# Autodesk Inventor assembly: OUTK_000_Assembly
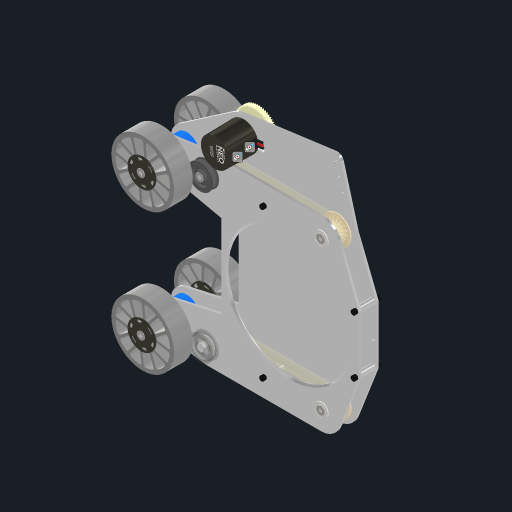
[picture p0: Inventor's stored thumbnail of the model, 512x512]
Saved by Autodesk Inventor 2024.2 (Build 282272000, 272)
## iProperties
Created: 2024-11-24
Part Number: OUTK_000_Assembly
Document SubType Name: Assembly
Designer: Bryan
Mass: 9682.5 g
Surface Area: 20203.5 cm^2
Volume: 5331.75 cm^3
Author: Bryan
## Documents named in this file (25)
- C:\Users\bobsb\OneDrive\Documents\GitHub\1622-2024-Casino-Clash-CAD-A-Thon\Outtake\OUTK_000_Assembly.iam
- C:\Users\bobsb\OneDrive\Documents\GitHub\1622-2024-Casino-Clash-CAD-A-Thon\Outtake\OUTK_002_ShotPlateNoReceptacle.ipt
- C:\Users\bobsb\OneDrive\Documents\GitHub\1622-2024-Casino-Clash-CAD-A-Thon\Outtake\OUTK_002_ShotPlateReceptacle.ipt
- C:\Users\bobsb\OneDrive\Documents\GitHub\1622-2024-Casino-Clash-CAD-A-Thon\COTS Library\Motion\Bearings\COTS_WCP-0783_1.125ODHexBearing.ipt
- C:\Users\bobsb\OneDrive\Documents\GitHub\1622-2024-Casino-Clash-CAD-A-Thon\COTS Library\Motion\Wheels\Compliant Wheels\5in compliant wheels\COTS_5 Straight Flex Wheel (.ipt
- C:\Users\bobsb\OneDrive\Documents\GitHub\1622-2024-Casino-Clash-CAD-A-Thon\COTS Library\Adapters\COTS_1_2” Hex Bore Aluminum VersaHub (217-2592)(1).ipt
- C:\Users\bobsb\OneDrive\Documents\GitHub\1622-2024-Casino-Clash-CAD-A-Thon\COTS Library\Motion\Wheels\Compliant Wheels\2in compliant wheels\0.500in hex bore\COTS_am-3462_2indiameter_0.500inhexbore_durometer50A_CompliantWheel.ipt
- C:\Users\bobsb\OneDrive\Documents\GitHub\1622-2024-Casino-Clash-CAD-A-Thon\Outtake\OUTK_010_Grippy.ipt
- C:\Users\bobsb\OneDrive\Documents\GitHub\1622-2024-Casino-Clash-CAD-A-Thon\Outtake\OUTK_011_Tubing.ipt
- C:\Users\bobsb\OneDrive\Documents\GitHub\1622-2024-Casino-Clash-CAD-A-Thon\COTS Library\Fasteners\Bolts\Set Screws\10-32\COTS_91375A446_Alloy Steel Cup-Point Set Screw.ipt
- C:\Users\bobsb\OneDrive\Documents\GitHub\1622-2024-Casino-Clash-CAD-A-Thon\COTS Library\Motion\Pulleys\HTD5M\10mm Wide\COTS_30T_WCP-0565.ipt
- C:\Users\bobsb\OneDrive\Documents\GitHub\1622-2024-Casino-Clash-CAD-A-Thon\COTS Library\Motors\COTS_REV-21-1650-V1.1_Neo1.1.ipt
- C:\Users\bobsb\OneDrive\Documents\GitHub\1622-2024-Casino-Clash-CAD-A-Thon\COTS Library\Fasteners\Bolts\Button-Head\10-32\COTS_91255A265_Button Head Hex Drive Screw.ipt
- C:\Users\bobsb\OneDrive\Documents\GitHub\1622-2024-Casino-Clash-CAD-A-Thon\COTS Library\Adapters\COTS_REV-21-1879_8mmKeyTo0.5Hex.ipt
- C:\Users\bobsb\OneDrive\Documents\GitHub\1622-2024-Casino-Clash-CAD-A-Thon\COTS Library\Motion\Pulleys\HTD5M\10mm Wide\COTS_24T_WCP-0564.ipt
- C:\Users\bobsb\OneDrive\Documents\GitHub\1622-2024-Casino-Clash-CAD-A-Thon\COTS Library\Motion\Gears\20DP gears\Aluminum\0.5in hex\COTS_60T_WCP-0720(1).ipt
- C:\Users\bobsb\OneDrive\Documents\GitHub\1622-2024-Casino-Clash-CAD-A-Thon\Outtake\OUTK_012_Spacer1.ipt
- C:\Users\bobsb\OneDrive\Documents\GitHub\1622-2024-Casino-Clash-CAD-A-Thon\Outtake\OUTK_013_Standoff1.ipt
- C:\Users\bobsb\OneDrive\Documents\GitHub\1622-2024-Casino-Clash-CAD-A-Thon\COTS Library\Fasteners\Bolts\Socket-Head\0.25-20\COTS_91251A537_Black-Oxide Alloy Steel Socket Head Screw_.25-20_.5in.ipt
- C:\Users\bobsb\OneDrive\Documents\GitHub\1622-2024-Casino-Clash-CAD-A-Thon\Outtake\OUTK_014_Shaft1.ipt
- C:\Users\bobsb\OneDrive\Documents\GitHub\1622-2024-Casino-Clash-CAD-A-Thon\Outtake\OUTK_015_Shaft2.ipt
- C:\Users\bobsb\OneDrive\Documents\GitHub\1622-2024-Casino-Clash-CAD-A-Thon\Outtake\OUTK_016_Shaft3.ipt
- C:\Users\bobsb\OneDrive\Documents\GitHub\1622-2024-Casino-Clash-CAD-A-Thon\Outtake\OUTK_016_Shaft4.ipt
- C:\Users\bobsb\OneDrive\Documents\GitHub\1622-2024-Casino-Clash-CAD-A-Thon\Outtake\OUTK_018_Spacer2.ipt
- C:\Users\bobsb\OneDrive\Documents\GitHub\1622-2024-Casino-Clash-CAD-A-Thon\COTS Library\Fasteners\Washers\COTS_90107A029_316 Stainless Steel Washer.ipt
## Components (131 placed, 24 different names)
1. OUTK_002_ShotPlateReceptacle:1 — Mate:141, Mate:179, Mate:183, Mate:185, Mate:190, Mate:205, Mate:207, Mate:208, Mate:210, Mate:211, Mate:212, Mate:213, Mate:225, Mate:228, Mate:229, Mate:232, Mate:244, Mate:245, Mate:246, Mate:247, Mate:249, Mate:251, Mate:252, Mate:253, Mate:254, Mate:255, Mate:262, Mate:267
2. COTS_WCP-0783_1.125ODHexBearing:1 — Mate:72, Mate:107, Mate:166, Mate:168, Mate:204
3. COTS_WCP-0783_1.125ODHexBearing:2 — Mate:74, Mate:106, Mate:108, Mate:145, Mate:205, Mate:208, Mate:235
4. COTS_WCP-0783_1.125ODHexBearing:3 — Mate:120, Mate:143, Mate:146, Mate:229, Mate:232
5. COTS_WCP-0783_1.125ODHexBearing:4 — Mate:124, Mate:230, Mate:231, Mate:269, Flush:24
6. COTS_WCP-0783_1.125ODHexBearing:5 — Mate:117, Mate:225, Mate:228, Flush:21
7. COTS_WCP-0783_1.125ODHexBearing:6 — Mate:123, Mate:226, Mate:227, Mate:258
8. COTS_WCP-0783_1.125ODHexBearing:7 — Mate:122, Mate:160, Mate:200, Mate:222
9. COTS_WCP-0783_1.125ODHexBearing:8 — Mate:71, Mate:110, Mate:111, Mate:163, Mate:165, Mate:215
10. COTS_WCP-0783_1.125ODHexBearing:9 — Mate:119, Mate:142, Mate:144, Mate:267
11. COTS_WCP-0783_1.125ODHexBearing:10 — Mate:73, Mate:112, Mate:139, Mate:140, Mate:207, Mate:213, Mate:214
12. COTS_WCP-0783_1.125ODHexBearing:11 — Mate:121, Mate:223, Mate:224
13. COTS_WCP-0783_1.125ODHexBearing:12 — Mate:118, Mate:197, Flush:18, Mate:262
14. COTS_5 Straight Flex Wheel (:1 — Mate:71, Mate:75, Mate:80, Mate:85, Mate:88, Mate:89, Mate:90
15. COTS_5 Straight Flex Wheel (:2 — Mate:72, Mate:76, Mate:81, Mate:86, Mate:87, Mate:94, Mate:95, Mate:96
16. COTS_5 Straight Flex Wheel (:3 — Mate:73, Mate:78, Mate:79, Mate:84, Mate:91, Mate:92, Mate:93
17. COTS_5 Straight Flex Wheel (:4 — Mate:74, Mate:77, Mate:82, Mate:83, Mate:97, Mate:98, Mate:99
18. COTS_1_2” Hex Bore Aluminum VersaHub (217-2592)(1):1 — Mate:77, Mate:82, Mate:83, Mate:135, Flush:8, Mate:194, Flush:14
19. COTS_1_2” Hex Bore Aluminum VersaHub (217-2592)(1):2 — Mate:76, Mate:81, Mate:86, Mate:87, Mate:130, Flush:3
20. COTS_1_2” Hex Bore Aluminum VersaHub (217-2592)(1):3 — Mate:78, Mate:79, Mate:84, Mate:134, Flush:7, Mate:193, Flush:13
21. COTS_1_2” Hex Bore Aluminum VersaHub (217-2592)(1):4 — Mate:75, Mate:80, Mate:85, Mate:131, Flush:4
22. COTS_1_2” Hex Bore Aluminum VersaHub (217-2592)(1):5 — Mate:88, Mate:89, Mate:90, Mate:132, Flush:5, Mate:164
23. COTS_1_2” Hex Bore Aluminum VersaHub (217-2592)(1):6 — Mate:91, Mate:92, Mate:93, Mate:133, Flush:6, Mate:147
24. COTS_1_2” Hex Bore Aluminum VersaHub (217-2592)(1):7 — Mate:94, Mate:95, Mate:96, Mate:129, Flush:2, Mate:167
25. COTS_1_2” Hex Bore Aluminum VersaHub (217-2592)(1):8 — Mate:97, Mate:98, Mate:99, Mate:136, Flush:9, Mate:148
26. COTS_am-3462_2indiameter_0.500inhexbore_durometer50A_CompliantWheel:1 — Mate:106, Mate:107, Mate:109, Mate:204
27. COTS_am-3462_2indiameter_0.500inhexbore_durometer50A_CompliantWheel:2 — Mate:108, Mate:109, Flush:20
28. COTS_am-3462_2indiameter_0.500inhexbore_durometer50A_CompliantWheel:3 — Mate:110, Mate:111, Mate:113, Mate:203, Flush:19
29. COTS_am-3462_2indiameter_0.500inhexbore_durometer50A_CompliantWheel:4 — Mate:112, Mate:113, Mate:203, Flush:20, Mate:214
30. OUTK_010_Grippy:1 — Mate:120, Mate:124, Mate:128
31. OUTK_010_Grippy:2 — Mate:119, Mate:122, Mate:126, Flush:19
32. OUTK_010_Grippy:3 — Mate:118, Mate:121, Mate:125, Tangent:4
33. OUTK_010_Grippy:4 — Mate:117, Mate:123, Mate:127, Tangent:5
34. OUTK_011_Tubing:1 — Mate:125, Mate:126, Tangent:4
35. OUTK_011_Tubing:2 — Mate:127, Mate:128, Tangent:5
36. COTS_30T_WCP-0565:1 — Mate:139, Mate:140, Mate:147
37. COTS_30T_WCP-0565:2 — Mate:141, Mate:145, Mate:148
38. COTS_30T_WCP-0565:3 — Mate:143, Mate:146
39. COTS_30T_WCP-0565:4 — Mate:142, Mate:144, Mate:195, Flush:15
40. COTS_REV-21-1879_8mmKeyTo0.5Hex:1 — Flush:11, Mate:219
41. COTS_24T_WCP-0564:1 — Mate:159, Mate:221, Flush:23
42. COTS_60T_WCP-0720(1):1 — Mate:159, Flush:11, Mate:220, Mate:264
43. COTS_60T_WCP-0720(1):2 — Mate:160, Mate:199, Mate:268
44. OUTK_012_Spacer1:1 — Mate:166, Mate:167, Mate:168
45. OUTK_012_Spacer1:2 — Mate:163, Mate:164, Mate:165
46. OUTK_013_Standoff1:1 — Mate:253, Mate:254
47. OUTK_013_Standoff1:2 — Mate:244, Mate:245
48. OUTK_013_Standoff1:3 — Mate:247, Mate:248
49. OUTK_013_Standoff1:4 — Mate:250, Mate:251
50. COTS_91251A537_Black-Oxide Alloy Steel Socket Head Screw_.25-20_.5in:1 — Mate:236, Mate:237, Mate:250
51. COTS_91251A537_Black-Oxide Alloy Steel Socket Head Screw_.25-20_.5in:2 — Mate:179, Mate:252
52. COTS_91251A537_Black-Oxide Alloy Steel Socket Head Screw_.25-20_.5in:3 — Mate:240, Mate:243
53. COTS_91251A537_Black-Oxide Alloy Steel Socket Head Screw_.25-20_.5in:4 — Mate:183, Mate:249
54. COTS_91251A537_Black-Oxide Alloy Steel Socket Head Screw_.25-20_.5in:5 — Mate:241, Mate:242
55. COTS_91251A537_Black-Oxide Alloy Steel Socket Head Screw_.25-20_.5in:6 — Mate:185, Mate:246
56. COTS_91251A537_Black-Oxide Alloy Steel Socket Head Screw_.25-20_.5in:7 — Mate:238, Mate:239
57. COTS_91251A537_Black-Oxide Alloy Steel Socket Head Screw_.25-20_.5in:8 — Mate:190, Mate:255
58. OUTK_014_Shaft1:1 — Mate:193, Flush:13, Mate:272, Mate:273, Mate:278, Mate:279
59. OUTK_015_Shaft2:1 — Mate:195, Flush:15, Mate:211, Mate:265, Mate:266, Mate:280, Mate:281
60. OUTK_016_Shaft4:1 — Mate:197, Flush:18, Mate:212, Mate:260, Mate:261, Mate:282, Mate:283
61. OUTK_014_Shaft1:2 — Mate:194, Flush:14, Mate:274, Mate:275, Mate:276, Mate:277
62. OUTK_018_Spacer2:1 — Mate:199, Mate:200, Mate:268
63. OUTK_002_ShotPlateNoReceptacle:1 — Mate:210, Mate:215, Mate:216, Mate:217, Mate:218, Mate:222, Mate:223, Mate:224, Mate:226, Mate:227, Mate:230, Mate:231, Mate:233, Mate:234, Mate:235, Mate:236, Mate:237, Mate:238, Mate:239, Mate:240, Mate:241, Mate:242, Mate:243, Mate:248
64. COTS_REV-21-1650-V1.1_Neo1.1:1 — Mate:216, Mate:217, Mate:218, Mate:219, Mate:220, Mate:221, Mate:263
65. COTS_24T_WCP-0564:3 — Mate:259, Flush:22, Flush:23
66. OUTK_016_Shaft3:2 — Mate:258, Flush:21, Mate:259, Flush:22, Mate:284, Mate:285
67. COTS_90107A029_316 Stainless Steel Washer:2
68. COTS_90107A029_316 Stainless Steel Washer:3 — Mate:260, Mate:261
69. COTS_90107A029_316 Stainless Steel Washer:4 — Mate:263, Mate:264
70. COTS_90107A029_316 Stainless Steel Washer:5 — Mate:265, Mate:266
71. OUTK_016_Shaft3:3 — Mate:269, Flush:24, Mate:270, Mate:271
72. COTS_90107A029_316 Stainless Steel Washer:6 — Mate:270, Mate:271
73. COTS_90107A029_316 Stainless Steel Washer:7 — Mate:272, Mate:273
74. COTS_90107A029_316 Stainless Steel Washer:8 — Mate:274, Mate:275
75. COTS_90107A029_316 Stainless Steel Washer:9 — Mate:276, Mate:277
76. COTS_90107A029_316 Stainless Steel Washer:10 — Mate:278, Mate:279
77. COTS_90107A029_316 Stainless Steel Washer:11 — Mate:280, Mate:281
78. COTS_90107A029_316 Stainless Steel Washer:12 — Mate:282, Mate:283
79. COTS_90107A029_316 Stainless Steel Washer:13 — Mate:284, Mate:285
80. COTS_91375A446_Alloy Steel Cup-Point Set Screw:13 — Mate:129, Flush:2
81. COTS_91375A446_Alloy Steel Cup-Point Set Screw:14
82. COTS_91375A446_Alloy Steel Cup-Point Set Screw:15
83. COTS_91375A446_Alloy Steel Cup-Point Set Screw:16
84. COTS_91375A446_Alloy Steel Cup-Point Set Screw:17
85. COTS_91375A446_Alloy Steel Cup-Point Set Screw:18
86. COTS_91375A446_Alloy Steel Cup-Point Set Screw:1 — Mate:130, Flush:3
87. COTS_91375A446_Alloy Steel Cup-Point Set Screw:19
88. COTS_91375A446_Alloy Steel Cup-Point Set Screw:20
89. COTS_91375A446_Alloy Steel Cup-Point Set Screw:21
90. COTS_91375A446_Alloy Steel Cup-Point Set Screw:22
91. COTS_91375A446_Alloy Steel Cup-Point Set Screw:23
92. COTS_91375A446_Alloy Steel Cup-Point Set Screw:6 — Mate:131, Flush:4
93. COTS_91375A446_Alloy Steel Cup-Point Set Screw:24
94. COTS_91375A446_Alloy Steel Cup-Point Set Screw:25
95. COTS_91375A446_Alloy Steel Cup-Point Set Screw:26
96. COTS_91375A446_Alloy Steel Cup-Point Set Screw:27
97. COTS_91375A446_Alloy Steel Cup-Point Set Screw:28
98. COTS_91375A446_Alloy Steel Cup-Point Set Screw:7 — Mate:132, Flush:5
99. COTS_91375A446_Alloy Steel Cup-Point Set Screw:29
100. COTS_91375A446_Alloy Steel Cup-Point Set Screw:30
101. COTS_91375A446_Alloy Steel Cup-Point Set Screw:31
102. COTS_91375A446_Alloy Steel Cup-Point Set Screw:32
103. COTS_91375A446_Alloy Steel Cup-Point Set Screw:33
104. COTS_91375A446_Alloy Steel Cup-Point Set Screw:11 — Mate:134, Flush:7
105. COTS_91375A446_Alloy Steel Cup-Point Set Screw:34
106. COTS_91375A446_Alloy Steel Cup-Point Set Screw:35
107. COTS_91375A446_Alloy Steel Cup-Point Set Screw:36
108. COTS_91375A446_Alloy Steel Cup-Point Set Screw:37
109. COTS_91375A446_Alloy Steel Cup-Point Set Screw:38
110. COTS_91375A446_Alloy Steel Cup-Point Set Screw:12 — Mate:133, Flush:6
111. COTS_91375A446_Alloy Steel Cup-Point Set Screw:39
112. COTS_91375A446_Alloy Steel Cup-Point Set Screw:40
113. COTS_91375A446_Alloy Steel Cup-Point Set Screw:41
114. COTS_91375A446_Alloy Steel Cup-Point Set Screw:42
115. COTS_91375A446_Alloy Steel Cup-Point Set Screw:43
116. COTS_91375A446_Alloy Steel Cup-Point Set Screw:9 — Mate:136, Flush:9
117. COTS_91375A446_Alloy Steel Cup-Point Set Screw:44
118. COTS_91375A446_Alloy Steel Cup-Point Set Screw:45
119. COTS_91375A446_Alloy Steel Cup-Point Set Screw:46
120. COTS_91375A446_Alloy Steel Cup-Point Set Screw:47
121. COTS_91375A446_Alloy Steel Cup-Point Set Screw:48
122. COTS_91375A446_Alloy Steel Cup-Point Set Screw:10 — Mate:135, Flush:8
123. COTS_91375A446_Alloy Steel Cup-Point Set Screw:49
124. COTS_91375A446_Alloy Steel Cup-Point Set Screw:50
125. COTS_91375A446_Alloy Steel Cup-Point Set Screw:51
126. COTS_91375A446_Alloy Steel Cup-Point Set Screw:52
127. COTS_91375A446_Alloy Steel Cup-Point Set Screw:53
128. COTS_91255A265_Button Head Hex Drive Screw:1 — Mate:233, Mate:234
129. COTS_91255A265_Button Head Hex Drive Screw:2
130. COTS_91255A265_Button Head Hex Drive Screw:3
131. COTS_91255A265_Button Head Hex Drive Screw:4
## Component patterns: (6 elements, first: COTS_91375A446_Alloy Steel Cup-Point Set Screw:13), (6 elements, first: COTS_91375A446_Alloy Steel Cup-Point Set Screw:1), (6 elements, first: COTS_91375A446_Alloy Steel Cup-Point Set Screw:6), (6 elements, first: COTS_91375A446_Alloy Steel Cup-Point Set Screw:7), (6 elements, first: COTS_91375A446_Alloy Steel Cup-Point Set Screw:11), (6 elements, first: COTS_91375A446_Alloy Steel Cup-Point Set Screw:12), (6 elements, first: COTS_91375A446_Alloy Steel Cup-Point Set Screw:9), (6 elements, first: COTS_91375A446_Alloy Steel Cup-Point Set Screw:10), (4 elements, first: COTS_91255A265_Button Head Hex Drive Screw:1)
## Relationships (188: Mate 166, Flush 19, Tangent 2, Angle 1)
- Mate:71: COTS_WCP-0783_1.125ODHexBearing:8 ↔ COTS_5 Straight Flex Wheel (:1
- Mate:72: COTS_WCP-0783_1.125ODHexBearing:1 ↔ COTS_5 Straight Flex Wheel (:2
- Mate:73: COTS_WCP-0783_1.125ODHexBearing:10 ↔ COTS_5 Straight Flex Wheel (:3
- Mate:74: COTS_WCP-0783_1.125ODHexBearing:2 ↔ COTS_5 Straight Flex Wheel (:4
- Mate:75: COTS_5 Straight Flex Wheel (:1 ↔ COTS_1_2” Hex Bore Aluminum VersaHub (217-2592)(1):4
- Mate:76: COTS_5 Straight Flex Wheel (:2 ↔ COTS_1_2” Hex Bore Aluminum VersaHub (217-2592)(1):2
- Mate:77: COTS_5 Straight Flex Wheel (:4 ↔ COTS_1_2” Hex Bore Aluminum VersaHub (217-2592)(1):1
- Mate:78: COTS_5 Straight Flex Wheel (:3 ↔ COTS_1_2” Hex Bore Aluminum VersaHub (217-2592)(1):3
- Mate:79: COTS_5 Straight Flex Wheel (:3 ↔ COTS_1_2” Hex Bore Aluminum VersaHub (217-2592)(1):3
- Mate:80: COTS_5 Straight Flex Wheel (:1 ↔ COTS_1_2” Hex Bore Aluminum VersaHub (217-2592)(1):4
- Mate:81: COTS_5 Straight Flex Wheel (:2 ↔ COTS_1_2” Hex Bore Aluminum VersaHub (217-2592)(1):2
- Mate:82: COTS_5 Straight Flex Wheel (:4 ↔ COTS_1_2” Hex Bore Aluminum VersaHub (217-2592)(1):1
- Mate:83: COTS_5 Straight Flex Wheel (:4 ↔ COTS_1_2” Hex Bore Aluminum VersaHub (217-2592)(1):1
- Mate:84: COTS_5 Straight Flex Wheel (:3 ↔ COTS_1_2” Hex Bore Aluminum VersaHub (217-2592)(1):3
- Mate:85: COTS_5 Straight Flex Wheel (:1 ↔ COTS_1_2” Hex Bore Aluminum VersaHub (217-2592)(1):4
- Mate:86: COTS_5 Straight Flex Wheel (:2 ↔ COTS_1_2” Hex Bore Aluminum VersaHub (217-2592)(1):2
- Mate:87: COTS_5 Straight Flex Wheel (:2 ↔ COTS_1_2” Hex Bore Aluminum VersaHub (217-2592)(1):2
- Mate:88: COTS_5 Straight Flex Wheel (:1 ↔ COTS_1_2” Hex Bore Aluminum VersaHub (217-2592)(1):5
- Mate:89: COTS_5 Straight Flex Wheel (:1 ↔ COTS_1_2” Hex Bore Aluminum VersaHub (217-2592)(1):5
- Mate:90: COTS_5 Straight Flex Wheel (:1 ↔ COTS_1_2” Hex Bore Aluminum VersaHub (217-2592)(1):5
- Mate:91: COTS_5 Straight Flex Wheel (:3 ↔ COTS_1_2” Hex Bore Aluminum VersaHub (217-2592)(1):6
- Mate:92: COTS_5 Straight Flex Wheel (:3 ↔ COTS_1_2” Hex Bore Aluminum VersaHub (217-2592)(1):6
- Mate:93: COTS_5 Straight Flex Wheel (:3 ↔ COTS_1_2” Hex Bore Aluminum VersaHub (217-2592)(1):6
- Mate:94: COTS_5 Straight Flex Wheel (:2 ↔ COTS_1_2” Hex Bore Aluminum VersaHub (217-2592)(1):7
- Mate:95: COTS_5 Straight Flex Wheel (:2 ↔ COTS_1_2” Hex Bore Aluminum VersaHub (217-2592)(1):7
- Mate:96: COTS_5 Straight Flex Wheel (:2 ↔ COTS_1_2” Hex Bore Aluminum VersaHub (217-2592)(1):7
- Mate:97: COTS_5 Straight Flex Wheel (:4 ↔ COTS_1_2” Hex Bore Aluminum VersaHub (217-2592)(1):8
- Mate:98: COTS_5 Straight Flex Wheel (:4 ↔ COTS_1_2” Hex Bore Aluminum VersaHub (217-2592)(1):8
- Mate:99: COTS_5 Straight Flex Wheel (:4 ↔ COTS_1_2” Hex Bore Aluminum VersaHub (217-2592)(1):8
- Mate:106: COTS_WCP-0783_1.125ODHexBearing:2 ↔ COTS_am-3462_2indiameter_0.500inhexbore_durometer50A_CompliantWheel:1
- Mate:107 (0.7937 mm): COTS_WCP-0783_1.125ODHexBearing:1 ↔ COTS_am-3462_2indiameter_0.500inhexbore_durometer50A_CompliantWheel:1
- Mate:108: COTS_WCP-0783_1.125ODHexBearing:2 ↔ COTS_am-3462_2indiameter_0.500inhexbore_durometer50A_CompliantWheel:2
- Mate:109: COTS_am-3462_2indiameter_0.500inhexbore_durometer50A_CompliantWheel:1 ↔ COTS_am-3462_2indiameter_0.500inhexbore_durometer50A_CompliantWheel:2
- Mate:110: COTS_WCP-0783_1.125ODHexBearing:8 ↔ COTS_am-3462_2indiameter_0.500inhexbore_durometer50A_CompliantWheel:3
- Mate:111 (0.7937 mm): COTS_WCP-0783_1.125ODHexBearing:8 ↔ COTS_am-3462_2indiameter_0.500inhexbore_durometer50A_CompliantWheel:3
- Mate:112: COTS_WCP-0783_1.125ODHexBearing:10 ↔ COTS_am-3462_2indiameter_0.500inhexbore_durometer50A_CompliantWheel:4
- Mate:113: COTS_am-3462_2indiameter_0.500inhexbore_durometer50A_CompliantWheel:3 ↔ COTS_am-3462_2indiameter_0.500inhexbore_durometer50A_CompliantWheel:4
- Mate:117: COTS_WCP-0783_1.125ODHexBearing:5 ↔ OUTK_010_Grippy:4
- Mate:118: COTS_WCP-0783_1.125ODHexBearing:12 ↔ OUTK_010_Grippy:3
- Mate:119: COTS_WCP-0783_1.125ODHexBearing:9 ↔ OUTK_010_Grippy:2
- Mate:120: COTS_WCP-0783_1.125ODHexBearing:3 ↔ OUTK_010_Grippy:1
- Mate:121 (0.7937 mm): COTS_WCP-0783_1.125ODHexBearing:11 ↔ OUTK_010_Grippy:3
- Mate:122 (0.7937 mm): COTS_WCP-0783_1.125ODHexBearing:7 ↔ OUTK_010_Grippy:2
- Mate:123 (0.7937 mm): COTS_WCP-0783_1.125ODHexBearing:6 ↔ OUTK_010_Grippy:4
- Mate:124 (0.7937 mm): COTS_WCP-0783_1.125ODHexBearing:4 ↔ OUTK_010_Grippy:1
- Mate:125: OUTK_010_Grippy:3 ↔ OUTK_011_Tubing:1
- Mate:126: OUTK_010_Grippy:2 ↔ OUTK_011_Tubing:1
- Tangent:4: OUTK_010_Grippy:3 ↔ OUTK_011_Tubing:1
- Mate:127: OUTK_010_Grippy:4 ↔ OUTK_011_Tubing:2
- Mate:128: OUTK_010_Grippy:1 ↔ OUTK_011_Tubing:2
- Tangent:5: OUTK_010_Grippy:4 ↔ OUTK_011_Tubing:2
- Mate:129: COTS_1_2” Hex Bore Aluminum VersaHub (217-2592)(1):7 ↔ COTS_91375A446_Alloy Steel Cup-Point Set Screw:13
- Flush:2: COTS_1_2” Hex Bore Aluminum VersaHub (217-2592)(1):7 ↔ COTS_91375A446_Alloy Steel Cup-Point Set Screw:13
- Mate:130: COTS_1_2” Hex Bore Aluminum VersaHub (217-2592)(1):2 ↔ COTS_91375A446_Alloy Steel Cup-Point Set Screw:1
- Flush:3: COTS_1_2” Hex Bore Aluminum VersaHub (217-2592)(1):2 ↔ COTS_91375A446_Alloy Steel Cup-Point Set Screw:1
- Mate:131: COTS_1_2” Hex Bore Aluminum VersaHub (217-2592)(1):4 ↔ COTS_91375A446_Alloy Steel Cup-Point Set Screw:6
- Flush:4: COTS_1_2” Hex Bore Aluminum VersaHub (217-2592)(1):4 ↔ COTS_91375A446_Alloy Steel Cup-Point Set Screw:6
- Mate:132: COTS_1_2” Hex Bore Aluminum VersaHub (217-2592)(1):5 ↔ COTS_91375A446_Alloy Steel Cup-Point Set Screw:7
- Flush:5: COTS_1_2” Hex Bore Aluminum VersaHub (217-2592)(1):5 ↔ COTS_91375A446_Alloy Steel Cup-Point Set Screw:7
- Mate:133: COTS_1_2” Hex Bore Aluminum VersaHub (217-2592)(1):6 ↔ COTS_91375A446_Alloy Steel Cup-Point Set Screw:12
- Flush:6: COTS_1_2” Hex Bore Aluminum VersaHub (217-2592)(1):6 ↔ COTS_91375A446_Alloy Steel Cup-Point Set Screw:12
- Mate:134: COTS_1_2” Hex Bore Aluminum VersaHub (217-2592)(1):3 ↔ COTS_91375A446_Alloy Steel Cup-Point Set Screw:11
- Flush:7: COTS_1_2” Hex Bore Aluminum VersaHub (217-2592)(1):3 ↔ COTS_91375A446_Alloy Steel Cup-Point Set Screw:11
- Mate:135: COTS_1_2” Hex Bore Aluminum VersaHub (217-2592)(1):1 ↔ COTS_91375A446_Alloy Steel Cup-Point Set Screw:10
- Flush:8: COTS_1_2” Hex Bore Aluminum VersaHub (217-2592)(1):1 ↔ COTS_91375A446_Alloy Steel Cup-Point Set Screw:10
- Mate:136: COTS_1_2” Hex Bore Aluminum VersaHub (217-2592)(1):8 ↔ COTS_91375A446_Alloy Steel Cup-Point Set Screw:9
- Flush:9: COTS_1_2” Hex Bore Aluminum VersaHub (217-2592)(1):8 ↔ COTS_91375A446_Alloy Steel Cup-Point Set Screw:9
- Mate:139: COTS_WCP-0783_1.125ODHexBearing:10 ↔ COTS_30T_WCP-0565:1
- Mate:140: COTS_WCP-0783_1.125ODHexBearing:10 ↔ COTS_30T_WCP-0565:1
- Mate:141: OUTK_002_ShotPlateReceptacle:1 ↔ COTS_30T_WCP-0565:2
- Mate:142: COTS_WCP-0783_1.125ODHexBearing:9 ↔ COTS_30T_WCP-0565:4
- Mate:143: COTS_WCP-0783_1.125ODHexBearing:3 ↔ COTS_30T_WCP-0565:3
- Mate:144: COTS_WCP-0783_1.125ODHexBearing:9 ↔ COTS_30T_WCP-0565:4
- Mate:145: COTS_WCP-0783_1.125ODHexBearing:2 ↔ COTS_30T_WCP-0565:2
- Mate:146: COTS_WCP-0783_1.125ODHexBearing:3 ↔ COTS_30T_WCP-0565:3
- Mate:147: COTS_1_2” Hex Bore Aluminum VersaHub (217-2592)(1):6 ↔ COTS_30T_WCP-0565:1
- Mate:148: COTS_1_2” Hex Bore Aluminum VersaHub (217-2592)(1):8 ↔ COTS_30T_WCP-0565:2
- Mate:159: COTS_24T_WCP-0564:1 ↔ COTS_60T_WCP-0720(1):1
- Flush:11: COTS_REV-21-1879_8mmKeyTo0.5Hex:1 ↔ COTS_60T_WCP-0720(1):1
- Mate:160: COTS_WCP-0783_1.125ODHexBearing:7 ↔ COTS_60T_WCP-0720(1):2
- Angle:1 (0 deg)
- Mate:163: COTS_WCP-0783_1.125ODHexBearing:8 ↔ OUTK_012_Spacer1:2
- Mate:164: COTS_1_2” Hex Bore Aluminum VersaHub (217-2592)(1):5 ↔ OUTK_012_Spacer1:2
- Mate:165: COTS_WCP-0783_1.125ODHexBearing:8 ↔ OUTK_012_Spacer1:2
- Mate:166: COTS_WCP-0783_1.125ODHexBearing:1 ↔ OUTK_012_Spacer1:1
- Mate:167: COTS_1_2” Hex Bore Aluminum VersaHub (217-2592)(1):7 ↔ OUTK_012_Spacer1:1
- Mate:168: COTS_WCP-0783_1.125ODHexBearing:1 ↔ OUTK_012_Spacer1:1
- Mate:179: OUTK_002_ShotPlateReceptacle:1 ↔ COTS_91251A537_Black-Oxide Alloy Steel Socket Head Screw_.25-20_.5in:2
- Mate:183: OUTK_002_ShotPlateReceptacle:1 ↔ COTS_91251A537_Black-Oxide Alloy Steel Socket Head Screw_.25-20_.5in:4
- Mate:185: OUTK_002_ShotPlateReceptacle:1 ↔ COTS_91251A537_Black-Oxide Alloy Steel Socket Head Screw_.25-20_.5in:6
- Mate:190: OUTK_002_ShotPlateReceptacle:1 ↔ COTS_91251A537_Black-Oxide Alloy Steel Socket Head Screw_.25-20_.5in:8
- Mate:193: COTS_1_2” Hex Bore Aluminum VersaHub (217-2592)(1):3 ↔ OUTK_014_Shaft1:1
- Flush:13: COTS_1_2” Hex Bore Aluminum VersaHub (217-2592)(1):3 ↔ OUTK_014_Shaft1:1
- Mate:194: COTS_1_2” Hex Bore Aluminum VersaHub (217-2592)(1):1 ↔ OUTK_014_Shaft1:2
- Flush:14: COTS_1_2” Hex Bore Aluminum VersaHub (217-2592)(1):1 ↔ OUTK_014_Shaft1:2
- Mate:195: COTS_30T_WCP-0565:4 ↔ OUTK_015_Shaft2:1
- Flush:15: COTS_30T_WCP-0565:4 ↔ OUTK_015_Shaft2:1
- Mate:197: COTS_WCP-0783_1.125ODHexBearing:12 ↔ OUTK_016_Shaft4:1
- Flush:18: COTS_WCP-0783_1.125ODHexBearing:12 ↔ OUTK_016_Shaft4:1
- Mate:199: COTS_60T_WCP-0720(1):2 ↔ OUTK_018_Spacer2:1
- Mate:200: COTS_WCP-0783_1.125ODHexBearing:7 ↔ OUTK_018_Spacer2:1
- Mate:203: COTS_am-3462_2indiameter_0.500inhexbore_durometer50A_CompliantWheel:3 ↔ COTS_am-3462_2indiameter_0.500inhexbore_durometer50A_CompliantWheel:4
- Flush:19: COTS_am-3462_2indiameter_0.500inhexbore_durometer50A_CompliantWheel:3 ↔ OUTK_010_Grippy:2
- Mate:204: COTS_WCP-0783_1.125ODHexBearing:1 ↔ COTS_am-3462_2indiameter_0.500inhexbore_durometer50A_CompliantWheel:1
- Mate:205: OUTK_002_ShotPlateReceptacle:1 ↔ COTS_WCP-0783_1.125ODHexBearing:2
- Mate:207: OUTK_002_ShotPlateReceptacle:1 ↔ COTS_WCP-0783_1.125ODHexBearing:10
- Mate:208: OUTK_002_ShotPlateReceptacle:1 ↔ COTS_WCP-0783_1.125ODHexBearing:2
- Flush:20: COTS_am-3462_2indiameter_0.500inhexbore_durometer50A_CompliantWheel:2 ↔ COTS_am-3462_2indiameter_0.500inhexbore_durometer50A_CompliantWheel:4
- Mate:210: OUTK_002_ShotPlateReceptacle:1 ↔ OUTK_002_ShotPlateNoReceptacle:1
- Mate:211: OUTK_002_ShotPlateReceptacle:1 ↔ OUTK_015_Shaft2:1
- Mate:212: OUTK_002_ShotPlateReceptacle:1 ↔ OUTK_016_Shaft4:1
- Mate:213: OUTK_002_ShotPlateReceptacle:1 ↔ COTS_WCP-0783_1.125ODHexBearing:10
- Mate:214 (0.7937 mm): COTS_WCP-0783_1.125ODHexBearing:10 ↔ COTS_am-3462_2indiameter_0.500inhexbore_durometer50A_CompliantWheel:4
- Mate:215: COTS_WCP-0783_1.125ODHexBearing:8 ↔ OUTK_002_ShotPlateNoReceptacle:1
- Mate:216: OUTK_002_ShotPlateNoReceptacle:1 ↔ COTS_REV-21-1650-V1.1_Neo1.1:1
- Mate:217: OUTK_002_ShotPlateNoReceptacle:1 ↔ COTS_REV-21-1650-V1.1_Neo1.1:1
- Mate:218: OUTK_002_ShotPlateNoReceptacle:1 ↔ COTS_REV-21-1650-V1.1_Neo1.1:1
- Mate:219: COTS_REV-21-1879_8mmKeyTo0.5Hex:1 ↔ COTS_REV-21-1650-V1.1_Neo1.1:1
- Mate:220: COTS_60T_WCP-0720(1):1 ↔ COTS_REV-21-1650-V1.1_Neo1.1:1
- Mate:221: COTS_24T_WCP-0564:1 ↔ COTS_REV-21-1650-V1.1_Neo1.1:1
- Mate:222: COTS_WCP-0783_1.125ODHexBearing:7 ↔ OUTK_002_ShotPlateNoReceptacle:1
- Mate:223: COTS_WCP-0783_1.125ODHexBearing:11 ↔ OUTK_002_ShotPlateNoReceptacle:1
- Mate:224: COTS_WCP-0783_1.125ODHexBearing:11 ↔ OUTK_002_ShotPlateNoReceptacle:1
- Mate:225: OUTK_002_ShotPlateReceptacle:1 ↔ COTS_WCP-0783_1.125ODHexBearing:5
- Mate:226: COTS_WCP-0783_1.125ODHexBearing:6 ↔ OUTK_002_ShotPlateNoReceptacle:1
- Mate:227: COTS_WCP-0783_1.125ODHexBearing:6 ↔ OUTK_002_ShotPlateNoReceptacle:1
- Mate:228: OUTK_002_ShotPlateReceptacle:1 ↔ COTS_WCP-0783_1.125ODHexBearing:5
- Mate:229: OUTK_002_ShotPlateReceptacle:1 ↔ COTS_WCP-0783_1.125ODHexBearing:3
- Mate:230: COTS_WCP-0783_1.125ODHexBearing:4 ↔ OUTK_002_ShotPlateNoReceptacle:1
- Mate:231: COTS_WCP-0783_1.125ODHexBearing:4 ↔ OUTK_002_ShotPlateNoReceptacle:1
- Mate:232: OUTK_002_ShotPlateReceptacle:1 ↔ COTS_WCP-0783_1.125ODHexBearing:3
- Mate:233: OUTK_002_ShotPlateNoReceptacle:1 ↔ COTS_91255A265_Button Head Hex Drive Screw:1
- Mate:234: OUTK_002_ShotPlateNoReceptacle:1 ↔ COTS_91255A265_Button Head Hex Drive Screw:1
- Mate:235: COTS_WCP-0783_1.125ODHexBearing:2 ↔ OUTK_002_ShotPlateNoReceptacle:1
- Mate:236: COTS_91251A537_Black-Oxide Alloy Steel Socket Head Screw_.25-20_.5in:1 ↔ OUTK_002_ShotPlateNoReceptacle:1
- Mate:237: COTS_91251A537_Black-Oxide Alloy Steel Socket Head Screw_.25-20_.5in:1 ↔ OUTK_002_ShotPlateNoReceptacle:1
- Mate:238: COTS_91251A537_Black-Oxide Alloy Steel Socket Head Screw_.25-20_.5in:7 ↔ OUTK_002_ShotPlateNoReceptacle:1
- Mate:239: COTS_91251A537_Black-Oxide Alloy Steel Socket Head Screw_.25-20_.5in:7 ↔ OUTK_002_ShotPlateNoReceptacle:1
- Mate:240: COTS_91251A537_Black-Oxide Alloy Steel Socket Head Screw_.25-20_.5in:3 ↔ OUTK_002_ShotPlateNoReceptacle:1
- Mate:241: COTS_91251A537_Black-Oxide Alloy Steel Socket Head Screw_.25-20_.5in:5 ↔ OUTK_002_ShotPlateNoReceptacle:1
- Mate:242: COTS_91251A537_Black-Oxide Alloy Steel Socket Head Screw_.25-20_.5in:5 ↔ OUTK_002_ShotPlateNoReceptacle:1
- Mate:243: COTS_91251A537_Black-Oxide Alloy Steel Socket Head Screw_.25-20_.5in:3 ↔ OUTK_002_ShotPlateNoReceptacle:1
- Mate:244: OUTK_002_ShotPlateReceptacle:1 ↔ OUTK_013_Standoff1:2
- Mate:245: OUTK_002_ShotPlateReceptacle:1 ↔ OUTK_013_Standoff1:2
- Mate:246: OUTK_002_ShotPlateReceptacle:1 ↔ COTS_91251A537_Black-Oxide Alloy Steel Socket Head Screw_.25-20_.5in:6
- Mate:247: OUTK_002_ShotPlateReceptacle:1 ↔ OUTK_013_Standoff1:3
- Mate:248: OUTK_013_Standoff1:3 ↔ OUTK_002_ShotPlateNoReceptacle:1
- Mate:249: OUTK_002_ShotPlateReceptacle:1 ↔ COTS_91251A537_Black-Oxide Alloy Steel Socket Head Screw_.25-20_.5in:4
- Mate:250: OUTK_013_Standoff1:4 ↔ COTS_91251A537_Black-Oxide Alloy Steel Socket Head Screw_.25-20_.5in:1
- Mate:251: OUTK_002_ShotPlateReceptacle:1 ↔ OUTK_013_Standoff1:4
- Mate:252: OUTK_002_ShotPlateReceptacle:1 ↔ COTS_91251A537_Black-Oxide Alloy Steel Socket Head Screw_.25-20_.5in:2
- Mate:253: OUTK_002_ShotPlateReceptacle:1 ↔ OUTK_013_Standoff1:1
- Mate:254: OUTK_002_ShotPlateReceptacle:1 ↔ OUTK_013_Standoff1:1
- Mate:255: OUTK_002_ShotPlateReceptacle:1 ↔ COTS_91251A537_Black-Oxide Alloy Steel Socket Head Screw_.25-20_.5in:8
- [Mate]: COTS_24T_WCP-0564:3 ↔ COTS_90107A029_316 Stainless Steel Washer:2
- [Mate]: COTS_24T_WCP-0564:3 ↔ COTS_90107A029_316 Stainless Steel Washer:2
- Mate:258: COTS_WCP-0783_1.125ODHexBearing:6 ↔ OUTK_016_Shaft3:2
- Flush:21: COTS_WCP-0783_1.125ODHexBearing:5 ↔ OUTK_016_Shaft3:2
- Mate:259: COTS_24T_WCP-0564:3 ↔ OUTK_016_Shaft3:2
- Flush:22: COTS_24T_WCP-0564:3 ↔ OUTK_016_Shaft3:2
- Flush:23: COTS_24T_WCP-0564:1 ↔ COTS_24T_WCP-0564:3
- Mate:260: OUTK_016_Shaft4:1 ↔ COTS_90107A029_316 Stainless Steel Washer:3
- Mate:261: OUTK_016_Shaft4:1 ↔ COTS_90107A029_316 Stainless Steel Washer:3
- Mate:262: OUTK_002_ShotPlateReceptacle:1 ↔ COTS_WCP-0783_1.125ODHexBearing:12
- Mate:263: COTS_REV-21-1650-V1.1_Neo1.1:1 ↔ COTS_90107A029_316 Stainless Steel Washer:4
- Mate:264: COTS_60T_WCP-0720(1):1 ↔ COTS_90107A029_316 Stainless Steel Washer:4
- Mate:265: OUTK_015_Shaft2:1 ↔ COTS_90107A029_316 Stainless Steel Washer:5
- Mate:266: OUTK_015_Shaft2:1 ↔ COTS_90107A029_316 Stainless Steel Washer:5
- Mate:267: OUTK_002_ShotPlateReceptacle:1 ↔ COTS_WCP-0783_1.125ODHexBearing:9
- Mate:268: COTS_60T_WCP-0720(1):2 ↔ OUTK_018_Spacer2:1
- Mate:269: COTS_WCP-0783_1.125ODHexBearing:4 ↔ OUTK_016_Shaft3:3
- Flush:24: COTS_WCP-0783_1.125ODHexBearing:4 ↔ OUTK_016_Shaft3:3
- Mate:270: OUTK_016_Shaft3:3 ↔ COTS_90107A029_316 Stainless Steel Washer:6
- Mate:271: OUTK_016_Shaft3:3 ↔ COTS_90107A029_316 Stainless Steel Washer:6
- Mate:272: OUTK_014_Shaft1:1 ↔ COTS_90107A029_316 Stainless Steel Washer:7
- Mate:273: OUTK_014_Shaft1:1 ↔ COTS_90107A029_316 Stainless Steel Washer:7
- Mate:274: OUTK_014_Shaft1:2 ↔ COTS_90107A029_316 Stainless Steel Washer:8
- Mate:275: OUTK_014_Shaft1:2 ↔ COTS_90107A029_316 Stainless Steel Washer:8
- Mate:276: OUTK_014_Shaft1:2 ↔ COTS_90107A029_316 Stainless Steel Washer:9
- Mate:277: OUTK_014_Shaft1:2 ↔ COTS_90107A029_316 Stainless Steel Washer:9
- Mate:278: OUTK_014_Shaft1:1 ↔ COTS_90107A029_316 Stainless Steel Washer:10
- Mate:279: OUTK_014_Shaft1:1 ↔ COTS_90107A029_316 Stainless Steel Washer:10
- Mate:280: OUTK_015_Shaft2:1 ↔ COTS_90107A029_316 Stainless Steel Washer:11
- Mate:281: OUTK_015_Shaft2:1 ↔ COTS_90107A029_316 Stainless Steel Washer:11
- Mate:282: OUTK_016_Shaft4:1 ↔ COTS_90107A029_316 Stainless Steel Washer:12
- Mate:283: OUTK_016_Shaft4:1 ↔ COTS_90107A029_316 Stainless Steel Washer:12
- Mate:284: OUTK_016_Shaft3:2 ↔ COTS_90107A029_316 Stainless Steel Washer:13
- Mate:285: OUTK_016_Shaft3:2 ↔ COTS_90107A029_316 Stainless Steel Washer:13
## Named parameters: d358_d298 = 0 mm, d359_d299 = 0 mm
